# Autodesk Inventor assembly: Crank sub-assembly
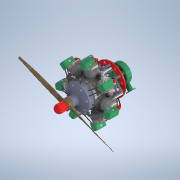
[picture p0: Inventor's stored thumbnail of the model, 180x180]
Saved by Autodesk Inventor 2021 (Build 250183000, 183)
## iProperties
Created: 2022-11-14
Part Number: Crank sub-assembly
Document SubType Name: Assembly
Designer: peris
Author: peris
## Documents named in this file (25)
- D:\Inventor\Radial_Engine\Assembly\Crank sub-assembly.iam
- D:\Inventor\Radial_Engine\Main_Block.ipt
- D:\Inventor\Radial_Engine\Assembly\Cylinder Complete.iam
- D:\Inventor\Radial_Engine\Assembly\mhxanh.iam
- C:\Users\peris\OneDrive\Έγγραφα\Inventor\Content Center Files\R2021\en-US\ISO 4762(1)\DIN EN ISO 4762 - M4 x 12.ipt
- D:\Inventor\Radial_Engine\Assembly\suction housing sub-assembly.iam
- D:\Inventor\Radial_Engine\Component 9.ipt
- D:\Inventor\Radial_Engine\Component 10.ipt
- D:\Inventor\Radial_Engine\Assembly\exhaust pipe sub assembly.iam
- D:\Inventor\Radial_Engine\Assembly\intake pipe sub assembly.iam
- D:\Inventor\Radial_Engine\Component 46.ipt
- C:\Users\peris\OneDrive\Έγγραφα\Inventor\Content Center Files\R2021\en-US\ISO 4762(2)\ISO 4762 - M3 x 5ISO.ipt
- C:\Users\peris\OneDrive\Έγγραφα\Inventor\Content Center Files\R2021\en-US\ISO 4762(2)\ISO 4762 - M3 x 10ISO.ipt
- C:\Users\peris\OneDrive\Έγγραφα\Inventor\Content Center Files\R2021\en-US\ISO 10511\ISO 10511 - M5.ipt
- D:\Inventor\Radial_Engine\Assembly\Cam Sub-assembly.iam
- D:\Inventor\Radial_Engine\Component 3.ipt
- D:\Inventor\Radial_Engine\Component 20.ipt
- C:\Users\peris\OneDrive\Έγγραφα\Inventor\Content Center Files\R2021\en-US\DIN 618 - T1  HK\DIN 618 - HK0609 - 6 x 10 x 9.ipt
- C:\Users\peris\OneDrive\Έγγραφα\Inventor\Content Center Files\R2021\en-US\DIN 6799\DIN 6799 - 6 7.ipt
- D:\Inventor\Radial_Engine\Assembly\Cam housing Sub-assembly.iam
- C:\Users\peris\OneDrive\Έγγραφα\Inventor\Content Center Files\R2021\en-US\ISO 4762(1)\DIN EN ISO 4762 - M3 x 25.ipt
- D:\Inventor\Radial_Engine\Component 43.ipt
- D:\Inventor\Radial_Engine\Component 42.ipt
- D:\Inventor\Radial_Engine\Component 44.ipt
- D:\Inventor\Radial_Engine\Component 53.ipt
## Components (128 placed, 24 different names)
1. Main_Block:1 — Flush:1, Flush:2, Mate:1, Mate:2, Mate:3, Mate:4, Mate:8, Mate:9, Mate:10, Mate:11, Mate:12, Mate:13, Mate:14, Mate:15, Mate:16, Mate:18, Mate:20, Mate:22, Mate:24, Mate:25, Mate:26, Mate:27, Mate:28, Mate:29, Mate:30, Mate:68, Mate:69, Mate:70, Mate:71, Mate:72, Mate:73, Mate:77, Mate:78, Mate:79, Mate:93, Mate:95, Mate:96
2. mhxanh:1 [sub-assembly] — Mate:6, Mate:7, Mate:8, Mate:9, Mate:10, Mate:11, Mate:12, Mate:13, Mate:14, Mate:92, Mate:94, Mate:113, Mate:116, Mate:120, Mate:121
3. suction housing sub-assembly:1 [sub-assembly] — Mate:24, Mate:25, Mate:26, Mate:27, Insert:1, Insert:2, Insert:3, Insert:4, Insert:5, Insert:6, Insert:7, Mate:61, Mate:62
4. Component 10:1 — Mate:30, Mate:31, Mate:32, Mate:47, Mate:60
5. Component 46:1 — Mate:47, Mate:48, Flush:3, Mate:49, Mate:50
6. ISO 4762 M3 x 10:1 — Insert:1
7. ISO 4762 M3 x 10:2 — Insert:2
8. ISO 4762 M3 x 10:3 — Insert:3
9. ISO 4762 M3 x 10:4 — Insert:4
10. ISO 4762 M3 x 10:5 — Insert:5
11. ISO 4762 M3 x 10:6 — Insert:6
12. ISO 4762 M3 x 10:7 — Insert:7
13. Cam Sub-assembly:1 [sub-assembly] — Mate:92, Mate:93, Tangent:1, Tangent:2, Tangent:3
14. Component 3:1 — Mate:70, Mate:73, Mate:76, Mate:84, Mate:85, Mate:86
15. Component 20:1 — Mate:75, Mate:77
16. Component 3:2 — Mate:68, Mate:71, Mate:74, Mate:82, Mate:83, Mate:90
17. Component 20:2 — Mate:74, Mate:78
18. Component 3:3 — Mate:69, Mate:72, Mate:75, Mate:80, Mate:81, Mate:88
19. Component 20:3 — Mate:76, Mate:79
20. DIN 618 - T1 HK HK0609 - 6 x 10 x 9:1 — Mate:80, Mate:81, Mate:89
21. DIN 618 - T1 HK HK0609 - 6 x 10 x 9:2 — Mate:82, Mate:83, Mate:91
22. DIN 618 - T1 HK HK0609 - 6 x 10 x 9:3 — Mate:84, Mate:85, Mate:87
23. DIN 6799 6:1 — Mate:86, Mate:87
24. DIN 6799 6:2 — Mate:88, Mate:89
25. DIN 6799 6:3 — Mate:90, Mate:91
26. Cam housing Sub-assembly:1 [sub-assembly] — Mate:94, Mate:95, Mate:96, Mate:97, Mate:98, Mate:99, Mate:100, Mate:101, Mate:102, Mate:103, Mate:104, Mate:105, Mate:106, Mate:107, Mate:108, Mate:109, Mate:110, Mate:111, Mate:112, Mate:114, Mate:117
27. DIN EN ISO 4762 M3 x 25:1 — Mate:99, Mate:100
28. DIN EN ISO 4762 M3 x 25:2 — Mate:101, Mate:102
29. DIN EN ISO 4762 M3 x 25:3 — Mate:103, Mate:104
30. DIN EN ISO 4762 M3 x 25:4 — Mate:105, Mate:106
31. DIN EN ISO 4762 M3 x 25:5 — Mate:107, Mate:108
32. DIN EN ISO 4762 M3 x 25:6 — Mate:109, Mate:110
33. DIN EN ISO 4762 M3 x 25:7 — Mate:111, Mate:112
34. Component 43:1 — Mate:113, Mate:114, Mate:115
35. Component 42:1 — Mate:116, Mate:117, Mate:122
36. Component 44:1 — Mate:120, Mate:123, Mate:124
37. Component 53:1 — Mate:121, Mate:122, Mate:123
38. Cylinder Complete:1 [sub-assembly] — Mate:2, Mate:3, Mate:4, Mate:6, Mate:7, Mate:15, Mate:17, Mate:19, Mate:21, Mate:23, Tangent:1, Tangent:2, Tangent:3, Mate:97, Mate:98
39. DIN EN ISO 4762 M4 x 12:1 — Mate:16, Mate:17
40. DIN EN ISO 4762 M4 x 12:3 — Mate:20, Mate:21
41. DIN EN ISO 4762 M4 x 12:4 — Mate:22, Mate:23
42. DIN EN ISO 4762 M4 x 12:2 — Mate:18, Mate:19
43. Cylinder Complete:2 [sub-assembly]
44. DIN EN ISO 4762 M4 x 12:5
45. DIN EN ISO 4762 M4 x 12:6
46. DIN EN ISO 4762 M4 x 12:7
47. DIN EN ISO 4762 M4 x 12:8
48. Cylinder Complete:3 [sub-assembly]
49. DIN EN ISO 4762 M4 x 12:9
50. DIN EN ISO 4762 M4 x 12:10
51. DIN EN ISO 4762 M4 x 12:11
52. DIN EN ISO 4762 M4 x 12:12
53. Cylinder Complete:4 [sub-assembly]
54. DIN EN ISO 4762 M4 x 12:13
55. DIN EN ISO 4762 M4 x 12:14
56. DIN EN ISO 4762 M4 x 12:15
57. DIN EN ISO 4762 M4 x 12:16
58. Cylinder Complete:5 [sub-assembly] — Mate:44, Mate:45, Mate:46, Mate:51, Mate:53, Flush:4, Mate:63, Mate:64, Mate:66
59. DIN EN ISO 4762 M4 x 12:17
60. DIN EN ISO 4762 M4 x 12:18
61. DIN EN ISO 4762 M4 x 12:19
62. DIN EN ISO 4762 M4 x 12:20
63. Cylinder Complete:6 [sub-assembly]
64. DIN EN ISO 4762 M4 x 12:21
65. DIN EN ISO 4762 M4 x 12:22
66. DIN EN ISO 4762 M4 x 12:23
67. DIN EN ISO 4762 M4 x 12:24
68. Cylinder Complete:7 [sub-assembly]
69. DIN EN ISO 4762 M4 x 12:25
70. DIN EN ISO 4762 M4 x 12:26
71. DIN EN ISO 4762 M4 x 12:27
72. DIN EN ISO 4762 M4 x 12:28
73. intake pipe sub assembly:1 [sub-assembly] — Mate:61, Flush:5, Mate:62, Mate:63, Mate:65, Mate:67
74. exhaust pipe sub assembly:1 [sub-assembly] — Mate:44, Mate:45, Mate:46, Mate:49, Mate:50, Mate:52, Mate:54
75. ISO 4762 M3 x 5:1 — Mate:51, Mate:52
76. ISO 4762 M3 x 5:2 — Mate:53, Mate:54
77. intake pipe sub assembly:2 [sub-assembly]
78. exhaust pipe sub assembly:2 [sub-assembly]
79. ISO 4762 M3 x 5:3
80. ISO 4762 M3 x 5:4
81. intake pipe sub assembly:3 [sub-assembly]
82. exhaust pipe sub assembly:3 [sub-assembly]
83. ISO 4762 M3 x 5:5
84. ISO 4762 M3 x 5:6
85. intake pipe sub assembly:4 [sub-assembly]
86. exhaust pipe sub assembly:4 [sub-assembly]
87. ISO 4762 M3 x 5:7
88. ISO 4762 M3 x 5:8
89. intake pipe sub assembly:5 [sub-assembly]
90. exhaust pipe sub assembly:5 [sub-assembly]
91. ISO 4762 M3 x 5:9
92. ISO 4762 M3 x 5:10
93. intake pipe sub assembly:6 [sub-assembly]
94. exhaust pipe sub assembly:6 [sub-assembly]
95. ISO 4762 M3 x 5:11
96. ISO 4762 M3 x 5:12
97. intake pipe sub assembly:7 [sub-assembly]
98. exhaust pipe sub assembly:7 [sub-assembly]
99. ISO 4762 M3 x 5:13
100. ISO 4762 M3 x 5:14
101. ISO 4762 M3 x 10:9 — Mate:66, Mate:67
102. ISO 4762 M3 x 10:8 — Mate:64, Mate:65
103. ISO 4762 M3 x 10:10
104. ISO 4762 M3 x 10:11
105. ISO 4762 M3 x 10:12
106. ISO 4762 M3 x 10:13
107. ISO 4762 M3 x 10:14
108. ISO 4762 M3 x 10:15
109. ISO 4762 M3 x 10:16
110. ISO 4762 M3 x 10:17
111. ISO 4762 M3 x 10:18
112. ISO 4762 M3 x 10:19
113. ISO 4762 M3 x 10:20
114. ISO 4762 M3 x 10:21
115. Component 9:1 — Mate:28, Mate:29, Mate:31, Mate:32, Mate:59
116. DIN EN ISO 10511 M5:1 — Mate:59, Mate:60
117. Component 9:2
118. DIN EN ISO 10511 M5:2
119. Component 9:3
120. DIN EN ISO 10511 M5:3
121. Component 9:4
122. DIN EN ISO 10511 M5:4
123. Component 9:5
124. DIN EN ISO 10511 M5:5
125. Component 9:6
126. DIN EN ISO 10511 M5:6
127. Component 9:7
128. DIN EN ISO 10511 M5:7
## Component patterns: (7 elements, first: Cylinder Complete:1 + DIN EN ISO 4762 M4 x 12:1 + DIN EN ISO 4762 M4 x 12:3 + DIN EN ISO 4762 M4 x 12:4 + DIN EN ISO 4762 M4 x 12:2), (7 elements, first: intake pipe sub assembly:1 + exhaust pipe sub assembly:1 + ISO 4762 M3 x 5:1 + ISO 4762 M3 x 5:2), (7 elements, first: ISO 4762 M3 x 10:9 + ISO 4762 M3 x 10:8), (7 elements, first: Component 9:1 + DIN EN ISO 10511 M5:1)
## Relationships (121: Mate 106, Insert 7, Flush 5, Tangent 3)
- Flush:1: Main_Block:1
- Flush:2: Main_Block:1
- Mate:1: Main_Block:1
- Mate:2: Main_Block:1 ↔ Cylinder Complete:1
- Mate:3: Main_Block:1 ↔ Cylinder Complete:1
- Mate:4: Main_Block:1 ↔ Cylinder Complete:1
- Mate:6: mhxanh:1 ↔ Cylinder Complete:1
- Mate:7: mhxanh:1 ↔ Cylinder Complete:1
- Mate:8: Main_Block:1 ↔ mhxanh:1
- Mate:9: Main_Block:1 ↔ mhxanh:1
- Mate:10: Main_Block:1 ↔ mhxanh:1
- Mate:11: Main_Block:1 ↔ mhxanh:1
- Mate:12: Main_Block:1 ↔ mhxanh:1
- Mate:13: Main_Block:1 ↔ mhxanh:1
- Mate:14: Main_Block:1 ↔ mhxanh:1
- Mate:15: Main_Block:1 ↔ Cylinder Complete:1
- Mate:16: Main_Block:1 ↔ DIN EN ISO 4762 M4 x 12:1
- Mate:17: Cylinder Complete:1 ↔ DIN EN ISO 4762 M4 x 12:1
- Mate:18: Main_Block:1 ↔ DIN EN ISO 4762 M4 x 12:2
- Mate:19: Cylinder Complete:1 ↔ DIN EN ISO 4762 M4 x 12:2
- Mate:20: Main_Block:1 ↔ DIN EN ISO 4762 M4 x 12:3
- Mate:21: Cylinder Complete:1 ↔ DIN EN ISO 4762 M4 x 12:3
- Mate:22: Main_Block:1 ↔ DIN EN ISO 4762 M4 x 12:4
- Mate:23: Cylinder Complete:1 ↔ DIN EN ISO 4762 M4 x 12:4
- Mate:24: Main_Block:1 ↔ suction housing sub-assembly:1
- Mate:25: Main_Block:1 ↔ suction housing sub-assembly:1
- Mate:26: Main_Block:1 ↔ suction housing sub-assembly:1
- Mate:27: Main_Block:1 ↔ suction housing sub-assembly:1
- Mate:28: Main_Block:1 ↔ Component 9:1
- Mate:29: Main_Block:1 ↔ Component 9:1
- Mate:30: Main_Block:1 ↔ Component 10:1
- Mate:31: Component 10:1 ↔ Component 9:1
- Mate:32: Component 10:1 ↔ Component 9:1
- Mate:44: Cylinder Complete:5 ↔ exhaust pipe sub assembly:1
- Mate:45: Cylinder Complete:5 ↔ exhaust pipe sub assembly:1
- Mate:46: Cylinder Complete:5 ↔ exhaust pipe sub assembly:1
- Mate:47: Component 10:1 ↔ Component 46:1
- Mate:48: Component 46:1
- Flush:3: Component 46:1
- Mate:49: Component 46:1 ↔ exhaust pipe sub assembly:1
- Mate:50: Component 46:1 ↔ exhaust pipe sub assembly:1
- Mate:51: Cylinder Complete:5 ↔ ISO 4762 M3 x 5:1
- Mate:52: exhaust pipe sub assembly:1 ↔ ISO 4762 M3 x 5:1
- Mate:53: Cylinder Complete:5 ↔ ISO 4762 M3 x 5:2
- Mate:54: exhaust pipe sub assembly:1 ↔ ISO 4762 M3 x 5:2
- Insert:1: suction housing sub-assembly:1 ↔ ISO 4762 M3 x 10:1
- Insert:2: suction housing sub-assembly:1 ↔ ISO 4762 M3 x 10:2
- Insert:3: suction housing sub-assembly:1 ↔ ISO 4762 M3 x 10:3
- Insert:4: suction housing sub-assembly:1 ↔ ISO 4762 M3 x 10:4
- Insert:5: suction housing sub-assembly:1 ↔ ISO 4762 M3 x 10:5
- Insert:6: suction housing sub-assembly:1 ↔ ISO 4762 M3 x 10:6
- Insert:7: suction housing sub-assembly:1 ↔ ISO 4762 M3 x 10:7
- Mate:59: Component 9:1 ↔ DIN EN ISO 10511 M5:1
- Mate:60: Component 10:1 ↔ DIN EN ISO 10511 M5:1
- Mate:61: suction housing sub-assembly:1 ↔ intake pipe sub assembly:1
- Flush:4: Cylinder Complete:5
- Flush:5: intake pipe sub assembly:1
- Mate:62: suction housing sub-assembly:1 ↔ intake pipe sub assembly:1
- Mate:63: Cylinder Complete:5 ↔ intake pipe sub assembly:1
- Mate:64: Cylinder Complete:5 ↔ ISO 4762 M3 x 10:8
- Mate:65: intake pipe sub assembly:1 ↔ ISO 4762 M3 x 10:8
- Mate:66: Cylinder Complete:5 ↔ ISO 4762 M3 x 10:9
- Mate:67: intake pipe sub assembly:1 ↔ ISO 4762 M3 x 10:9
- Mate:68: Main_Block:1 ↔ Component 3:2
- Mate:69: Main_Block:1 ↔ Component 3:3
- Mate:70: Main_Block:1 ↔ Component 3:1
- Mate:71: Main_Block:1 ↔ Component 3:2
- Mate:72: Main_Block:1 ↔ Component 3:3
- Mate:73: Main_Block:1 ↔ Component 3:1
- Mate:74: Component 3:2 ↔ Component 20:2
- Mate:75: Component 20:1 ↔ Component 3:3
- Mate:76: Component 3:1 ↔ Component 20:3
- Mate:77: Main_Block:1 ↔ Component 20:1
- Mate:78: Main_Block:1 ↔ Component 20:2
- Mate:79: Main_Block:1 ↔ Component 20:3
- Mate:80: Component 3:3 ↔ DIN 618 - T1 HK HK0609 - 6 x 10 x 9:1
- Mate:81: Component 3:3 ↔ DIN 618 - T1 HK HK0609 - 6 x 10 x 9:1
- Mate:82: Component 3:2 ↔ DIN 618 - T1 HK HK0609 - 6 x 10 x 9:2
- Mate:83: Component 3:2 ↔ DIN 618 - T1 HK HK0609 - 6 x 10 x 9:2
- Mate:84: Component 3:1 ↔ DIN 618 - T1 HK HK0609 - 6 x 10 x 9:3
- Mate:85: Component 3:1 ↔ DIN 618 - T1 HK HK0609 - 6 x 10 x 9:3
- Mate:86: Component 3:1 ↔ DIN 6799 6:1
- Mate:87: DIN 618 - T1 HK HK0609 - 6 x 10 x 9:3 ↔ DIN 6799 6:1
- Mate:88: Component 3:3 ↔ DIN 6799 6:2
- Mate:89: DIN 618 - T1 HK HK0609 - 6 x 10 x 9:1 ↔ DIN 6799 6:2
- Mate:90: Component 3:2 ↔ DIN 6799 6:3
- Mate:91: DIN 618 - T1 HK HK0609 - 6 x 10 x 9:2 ↔ DIN 6799 6:3
- Mate:92: mhxanh:1 ↔ Cam Sub-assembly:1
- Mate:93: Main_Block:1 ↔ Cam Sub-assembly:1
- Tangent:1: Cam Sub-assembly:1 ↔ Cylinder Complete:1
- Tangent:2: Cam Sub-assembly:1 ↔ Cylinder Complete:1
- Tangent:3: Cam Sub-assembly:1 ↔ Cylinder Complete:1
- Mate:94: mhxanh:1 ↔ Cam housing Sub-assembly:1
- Mate:95: Main_Block:1 ↔ Cam housing Sub-assembly:1
- Mate:96: Main_Block:1 ↔ Cam housing Sub-assembly:1
- Mate:97: Cam housing Sub-assembly:1 ↔ Cylinder Complete:1
- Mate:98: Cam housing Sub-assembly:1 ↔ Cylinder Complete:1
- Mate:99: Cam housing Sub-assembly:1 ↔ DIN EN ISO 4762 M3 x 25:1
- Mate:100: Cam housing Sub-assembly:1 ↔ DIN EN ISO 4762 M3 x 25:1
- Mate:101: Cam housing Sub-assembly:1 ↔ DIN EN ISO 4762 M3 x 25:2
- Mate:102: Cam housing Sub-assembly:1 ↔ DIN EN ISO 4762 M3 x 25:2
- Mate:103: Cam housing Sub-assembly:1 ↔ DIN EN ISO 4762 M3 x 25:3
- Mate:104: Cam housing Sub-assembly:1 ↔ DIN EN ISO 4762 M3 x 25:3
- Mate:105: Cam housing Sub-assembly:1 ↔ DIN EN ISO 4762 M3 x 25:4
- Mate:106: Cam housing Sub-assembly:1 ↔ DIN EN ISO 4762 M3 x 25:4
- Mate:107: Cam housing Sub-assembly:1 ↔ DIN EN ISO 4762 M3 x 25:5
- Mate:108: Cam housing Sub-assembly:1 ↔ DIN EN ISO 4762 M3 x 25:5
- Mate:109: Cam housing Sub-assembly:1 ↔ DIN EN ISO 4762 M3 x 25:6
- Mate:110: Cam housing Sub-assembly:1 ↔ DIN EN ISO 4762 M3 x 25:6
- Mate:111: Cam housing Sub-assembly:1 ↔ DIN EN ISO 4762 M3 x 25:7
- Mate:112: Cam housing Sub-assembly:1 ↔ DIN EN ISO 4762 M3 x 25:7
- Mate:113: mhxanh:1 ↔ Component 43:1
- Mate:114: Cam housing Sub-assembly:1 ↔ Component 43:1
- Mate:115: Component 43:1
- Mate:116: mhxanh:1 ↔ Component 42:1
- Mate:117: Cam housing Sub-assembly:1 ↔ Component 42:1
- Mate:120: mhxanh:1 ↔ Component 44:1
- Mate:121: mhxanh:1 ↔ Component 53:1
- Mate:122: Component 42:1 ↔ Component 53:1
- Mate:123: Component 44:1 ↔ Component 53:1
- Mate:124: Component 44:1
